# Autodesk Inventor assembly: pto piston
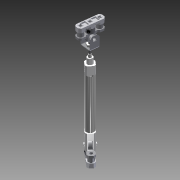
[picture p0: Inventor's stored thumbnail of the model, 180x180]
Saved by Autodesk Inventor 2014 SP1 (Build 180222100, 222)
## iProperties
Created: 2014-03-11
Part Number: pto piston
Document SubType Name: Assembly
Designer: Ryan
Author: Ryan
## Documents named in this file (8)
- C:\Users\Ryan\Desktop\sw\toss up 4th robot\drive\pto piston.iam
- C:\Users\Ryan\Desktop\sw\lib\Aperture VEX CAD Library\Bearing Blocks\Bearing Block.ipt
- C:\Users\Ryan\Desktop\sw\lib\Aperture VEX CAD Library\Hardware\Shaft Collar.ipt
- C:\Users\Ryan\Desktop\sw\lib\Aperture VEX CAD Library\Spacers\thin\SPACER-0320-0250.ipt
- C:\Users\Ryan\Desktop\sw\lib\Aperture VEX CAD Library\Bearing Blocks\Pillow Block.ipt
- C:\Users\Ryan\Desktop\sw\lib\Aperture VEX CAD Library\Pnuematics\End Gusset Fixed.ipt
- C:\Users\Ryan\Desktop\sw\lib\Aperture VEX CAD Library\Pnuematics\Cylinder, Bi-directional.iam
- C:\Users\Ryan\Desktop\sw\lib\Aperture VEX CAD Library\Pnuematics\Cylinder, Bi-directional-Parts\Nut 8-32 Hex.ipt
## Components (15 placed, 7 different names)
1. Bearing Block:1 — Mate:3, Mate:4, Mate:5, Mate:6, Mate:7, Mate:9
2. Shaft Collar:1 — Mate:5, Mate:9
3. SPACER-0320-0250:1 — Mate:1, Mate:2, Mate:3, Mate:4
4. SPACER-0320-0250:2 — Mate:6, Mate:7, Mate:8
5. Pillow Block:1 — Mate:1, Mate:2, Mate:8, Mate:10, Mate:21, Angle:2
6. SPACER-0320-0250:3 — Mate:14, Mate:15, Mate:19
7. SPACER-0320-0250:4 — Mate:10, Mate:11, Mate:13, Mate:15
8. End Gusset Fixed:1 — Mate:11, Mate:12, Mate:13, Mate:14, Mate:16, Mate:18, Mate:19, Mate:20, Angle:2
9. Cylinder, Bi-directional:1 [sub-assembly] — Mate:12, Mate:16, Mate:17, Mate:20, Mate:21, Mate:22, Mate:32, Angle:1
10. Nut 8-32 Hex:1 — Mate:17, Mate:18
11. Pillow Block:2 — Mate:22, Mate:23, Mate:24, Mate:31, Mate:32, Angle:1
12. SPACER-0320-0250:5 — Mate:29, Mate:30, Mate:31
13. Shaft Collar:2 — Mate:27, Mate:28
14. SPACER-0320-0250:6 — Mate:23, Mate:24, Mate:25, Mate:26
15. Bearing Block:2 — Mate:25, Mate:26, Mate:27, Mate:28, Mate:29, Mate:30
## Relationships (34: Mate 32, Angle 2)
- Mate:1: SPACER-0320-0250:1 ↔ Pillow Block:1
- Mate:2: SPACER-0320-0250:1 ↔ Pillow Block:1
- Mate:3: Bearing Block:1 ↔ SPACER-0320-0250:1
- Mate:4: Bearing Block:1 ↔ SPACER-0320-0250:1
- Mate:5: Bearing Block:1 ↔ Shaft Collar:1
- Mate:6: Bearing Block:1 ↔ SPACER-0320-0250:2
- Mate:7: Bearing Block:1 ↔ SPACER-0320-0250:2
- Mate:8: SPACER-0320-0250:2 ↔ Pillow Block:1
- Mate:9: Bearing Block:1 ↔ Shaft Collar:1
- Mate:10: Pillow Block:1 ↔ SPACER-0320-0250:4
- Mate:11: SPACER-0320-0250:4 ↔ End Gusset Fixed:1
- Mate:12 (2.3114 mm): End Gusset Fixed:1 ↔ Cylinder, Bi-directional:1
- Mate:13 (2.3114 mm): SPACER-0320-0250:4 ↔ End Gusset Fixed:1
- Mate:14: SPACER-0320-0250:3 ↔ End Gusset Fixed:1
- Mate:15: SPACER-0320-0250:3 ↔ SPACER-0320-0250:4
- Mate:16 (2.3114 mm): End Gusset Fixed:1 ↔ Cylinder, Bi-directional:1
- Mate:17: Cylinder, Bi-directional:1 ↔ Nut 8-32 Hex:1
- Mate:18: End Gusset Fixed:1 ↔ Nut 8-32 Hex:1
- Mate:19 (2.3114 mm): SPACER-0320-0250:3 ↔ End Gusset Fixed:1
- Mate:20: End Gusset Fixed:1 ↔ Cylinder, Bi-directional:1
- Mate:21: Pillow Block:1 ↔ Cylinder, Bi-directional:1
- Mate:22: Cylinder, Bi-directional:1 ↔ Pillow Block:2
- Mate:23: Pillow Block:2 ↔ SPACER-0320-0250:6
- Mate:24: Pillow Block:2 ↔ SPACER-0320-0250:6
- Mate:25: SPACER-0320-0250:6 ↔ Bearing Block:2
- Mate:26: SPACER-0320-0250:6 ↔ Bearing Block:2
- Mate:27: Shaft Collar:2 ↔ Bearing Block:2
- Mate:28: Shaft Collar:2 ↔ Bearing Block:2
- Mate:29: SPACER-0320-0250:5 ↔ Bearing Block:2
- Mate:30: SPACER-0320-0250:5 ↔ Bearing Block:2
- Mate:31: Pillow Block:2 ↔ SPACER-0320-0250:5
- Mate:32 (2.3876 mm): Cylinder, Bi-directional:1 ↔ Pillow Block:2
- Angle:1 (90 deg): Cylinder, Bi-directional:1 ↔ Pillow Block:2
- Angle:2 (90 deg): Pillow Block:1 ↔ End Gusset Fixed:1
## Named parameters: q = 2.3114 mm
